# Autodesk Inventor assembly: Assemblage absorbeur
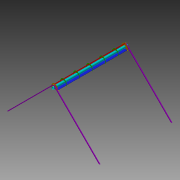
[picture p0: Inventor's stored thumbnail of the model, 180x180]
Saved by Autodesk Inventor 2015 SP1 (Build 190203100, 203)
## iProperties
Created: 2015-05-01
Part Number: Assemblage absorbeur
Document SubType Name: Assembly
Designer: Cyril
Author: Cyril
## Documents named in this file (9)
- C:\Users\Cyril\Documents\OSE FR\Concentrateur solaire\Inventor\Absorbeur\Assemblage absorbeur N-S.iam
- C:\Users\Cyril\Documents\OSE FR\Concentrateur solaire\Inventor\Absorbeur\Poutre centrale.ipt
- C:\Users\Cyril\Documents\OSE FR\Concentrateur solaire\Inventor\Absorbeur\Patron.ipt
- C:\Users\Cyril\Documents\OSE FR\Concentrateur solaire\Inventor\Absorbeur\Bouchon.ipt
- C:\Users\Cyril\Documents\OSE FR\Concentrateur solaire\Inventor\Absorbeur\Raccord.ipt
- C:\Users\Cyril\Documents\OSE FR\Concentrateur solaire\Inventor\Absorbeur\Pied.ipt
- C:\Users\Cyril\Documents\OSE FR\Concentrateur solaire\Inventor\Absorbeur\Vitre.ipt
- C:\Users\Cyril\Documents\OSE FR\Concentrateur solaire\Inventor\Absorbeur\Tube.ipt
- C:\Users\Cyril\Documents\OSE FR\Concentrateur solaire\Inventor\Absorbeur\Pied_MIR.ipt
## Components (16 placed, 8 different names)
1. Poutre centrale:1 — Mate:1, Mate:2, Mate:3, Mate:4, Mate:9, Mate:10, Angle:1, Mate:15, Mate:16, Mate:17, Mate:18, Mate:25, Mate:26, Mate:29, Mate:30
2. Bouchon:1 — Mate:29, Mate:30, Mate:31, Mate:33
3. Bouchon:2 — Mate:25, Mate:26, Mate:32
4. Raccord:1 — Mate:9, Mate:10, Mate:18
5. Raccord:2 — Mate:15, Mate:16, Mate:17, Mate:19, Mate:20, Mate:21, Mate:22, Mate:23, Mate:24
6. Pied:1 — Mate:19, Mate:20, Mate:21
7. Pied:2 — Mate:22, Mate:23, Mate:24
8. Vitre:1 — Mate:27, Mate:28, Mate:31, Mate:32
9. Tube:1 — Mate:33
10. Pied_MIR:1
11. Pied_MIR:2
12. Patron:1 — Mate:3, Mate:4
13. Patron:2
14. Patron:3
15. Patron:4
16. Patron:5 — Mate:28
## Component patterns: (5 elements, first: Patron:1)
## Relationships (26: Mate 25, Angle 1)
- Mate:1: Poutre centrale:1
- Mate:2: Poutre centrale:1
- Mate:3: Poutre centrale:1 ↔ Patron:1
- Mate:4: Poutre centrale:1 ↔ Patron:1
- Mate:9: Poutre centrale:1 ↔ Raccord:1
- Mate:10: Poutre centrale:1 ↔ Raccord:1
- Angle:1 (45 deg): Poutre centrale:1
- Mate:15: Poutre centrale:1 ↔ Raccord:2
- Mate:16: Poutre centrale:1 ↔ Raccord:2
- Mate:17: Poutre centrale:1 ↔ Raccord:2
- Mate:18: Poutre centrale:1 ↔ Raccord:1
- Mate:19: Raccord:2 ↔ Pied:1
- Mate:20: Raccord:2 ↔ Pied:1
- Mate:21: Raccord:2 ↔ Pied:1
- Mate:22: Raccord:2 ↔ Pied:2
- Mate:23: Raccord:2 ↔ Pied:2
- Mate:24: Raccord:2 ↔ Pied:2
- Mate:25: Poutre centrale:1 ↔ Bouchon:2
- Mate:26: Poutre centrale:1 ↔ Bouchon:2
- Mate:27: Vitre:1
- Mate:28: Vitre:1 ↔ Patron:5
- Mate:29: Poutre centrale:1 ↔ Bouchon:1
- Mate:30: Poutre centrale:1 ↔ Bouchon:1
- Mate:31 (5 mm): Bouchon:1 ↔ Vitre:1
- Mate:32 (5 mm): Bouchon:2 ↔ Vitre:1
- Mate:33: Bouchon:1 ↔ Tube:1
